# Autodesk Inventor assembly: Power Entry Module - Soanar PP4003
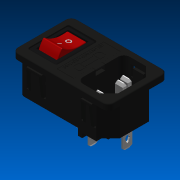
[picture p0: Inventor's stored thumbnail of the model, 180x180]
Saved by Autodesk Inventor 2016 (Build 200138000, 138)
## iProperties
Created: 2013-08-06
Document SubType Name: Assembly
Designer: sdarley
Project: Power Entry Module - Soanar PP4003
Catalog Web Link: https://www.soanarplus.com/getProductWebDetails.do?prodId=PP4003
Description: POWER ENTRY MODULE - SOANAR PP4003
Vendor: Soanar
Stock Number: PP4003
Author: sdarley
Title: Power Entry Module - Soanar PP4003
Revision Number: 1
## Documents named in this file (10)
- C:\Users\PowerStation9000\AppData\Local\Autodesk\Autodesk Sync\Cloud\mathiaslk\UltiBot mk2 rev2\Importerede komponenter\Power connector\Power Entry Module - Soanar PP4003.iam
- C:\Users\PowerStation9000\AppData\Local\Autodesk\Autodesk Sync\Cloud\mathiaslk\UltiBot mk2 rev2\Importerede komponenter\Power connector\Components\Rocker Switch - Arcolectric H8550VB\Rocker Switch - Arcolectric H8550VB.iam
- C:\Users\PowerStation9000\AppData\Local\Autodesk\Autodesk Sync\Cloud\mathiaslk\UltiBot mk2 rev2\Importerede komponenter\Power connector\Components\Soanar Power Module Fuse Cover.ipt
- C:\Users\PowerStation9000\AppData\Local\Autodesk\Autodesk Sync\Cloud\mathiaslk\UltiBot mk2 rev2\Importerede komponenter\Power connector\Components\Soanar Power Module Housing.ipt
- C:\Users\PowerStation9000\AppData\Local\Autodesk\Autodesk Sync\Cloud\mathiaslk\UltiBot mk2 rev2\Importerede komponenter\Power connector\Components\Soanar Power Module Pin A.ipt
- C:\Users\PowerStation9000\AppData\Local\Autodesk\Autodesk Sync\Cloud\mathiaslk\UltiBot mk2 rev2\Importerede komponenter\Power connector\Components\Soanar Power Module Pin B.ipt
- C:\Users\PowerStation9000\AppData\Local\Autodesk\Autodesk Sync\Cloud\mathiaslk\UltiBot mk2 rev2\Importerede komponenter\Power connector\Components\Soanar Power Module Pin C.ipt
- C:\Users\PowerStation9000\AppData\Local\Autodesk\Autodesk Sync\Cloud\mathiaslk\UltiBot mk2 rev2\Importerede komponenter\Power connector\Components\Soanar Power Module Pin D.ipt
- C:\Users\PowerStation9000\AppData\Local\Autodesk\Autodesk Sync\Cloud\mathiaslk\UltiBot mk2 rev2\Importerede komponenter\Power connector\Components\Soanar Power Module Pin E.ipt
- C:\Users\PowerStation9000\AppData\Local\Autodesk\Autodesk Sync\Cloud\mathiaslk\UltiBot mk2 rev2\Importerede komponenter\Power connector\Components\Soanar Power Module Fuse Holder.ipt
## Components (12 placed, 9 different names)
1. Soanar Power Module Housing:1 — Mate:1, Flush:1, Flush:2, Mate:4, Flush:4, Flush:5, Mate:2, Mate:5, Flush:6, Flush:7, Mate:6, Mate:7, Mate:8, Flush:8, Mate:12, Flush:14, Mate:14, Mate:16, Flush:15, Flush:16, Mate:20, Mate:22, Mate:23
2. Soanar Power Module Fuse Cover:1 — Flush:4, Flush:5, Mate:2, Mate:24, Mate:25, Mate:26
3. Soanar Power Module Pin A:1 — Flush:6, Flush:7, Mate:6, Mate:11
4. Soanar Power Module Pin B:1 — Mate:8, Mate:9, Mate:10, Mate:11, Flush:8
5. Soanar Power Module Pin B:2 — Mate:7, Mate:9, Mate:10
6. Soanar Power Module Pin C:1 — Mate:15, Mate:16, Mate:17, Mate:18, Mate:19
7. Soanar Power Module Pin C:2 — Mate:12, Flush:14, Mate:14, Mate:15, Mate:17, Flush:17, Mate:21
8. Soanar Power Module Pin D:1 — Flush:15, Mate:18, Mate:19
9. Soanar Power Module Pin E:1 — Flush:16, Mate:20, Flush:17
10. Soanar Power Module Fuse Holder:1 — Mate:23, Mate:24, Flush:18, Mate:26
11. Soanar Power Module Fuse Holder:2 — Mate:22, Mate:25, Flush:18
12. Rocker Switch - Arcolectric H8550VB:1 [sub-assembly] — Mate:1, Mate:4, Mate:5
## Relationships (36: Mate 24, Flush 12)
- Mate:1: Soanar Power Module Housing:1 ↔ Rocker Switch - Arcolectric H8550VB:1
- Flush:1: Soanar Power Module Housing:1
- Flush:2: Soanar Power Module Housing:1
- Mate:4: Soanar Power Module Housing:1 ↔ Rocker Switch - Arcolectric H8550VB:1
- Flush:4: Soanar Power Module Housing:1 ↔ Soanar Power Module Fuse Cover:1
- Flush:5: Soanar Power Module Housing:1 ↔ Soanar Power Module Fuse Cover:1
- Mate:2: Soanar Power Module Housing:1 ↔ Soanar Power Module Fuse Cover:1
- Mate:5 (0.025 mm): Soanar Power Module Housing:1 ↔ Rocker Switch - Arcolectric H8550VB:1
- Flush:6: Soanar Power Module Housing:1 ↔ Soanar Power Module Pin A:1
- Flush:7: Soanar Power Module Housing:1 ↔ Soanar Power Module Pin A:1
- Mate:6 (3.85 mm): Soanar Power Module Housing:1 ↔ Soanar Power Module Pin A:1
- Mate:7: Soanar Power Module Housing:1 ↔ Soanar Power Module Pin B:2
- Mate:8: Soanar Power Module Housing:1 ↔ Soanar Power Module Pin B:1
- Mate:9: Soanar Power Module Pin B:1 ↔ Soanar Power Module Pin B:2
- Mate:10 (13.15 mm): Soanar Power Module Pin B:1 ↔ Soanar Power Module Pin B:2
- Mate:11: Soanar Power Module Pin A:1 ↔ Soanar Power Module Pin B:1
- Flush:8 (-6.575 mm): Soanar Power Module Housing:1 ↔ Soanar Power Module Pin B:1
- Mate:12: Soanar Power Module Housing:1 ↔ Soanar Power Module Pin C:2
- Flush:14 (3.45 mm): Soanar Power Module Housing:1 ↔ Soanar Power Module Pin C:2
- Mate:14: Soanar Power Module Housing:1 ↔ Soanar Power Module Pin C:2
- Mate:15 (-11.2 mm): Soanar Power Module Pin C:1 ↔ Soanar Power Module Pin C:2
- Mate:16: Soanar Power Module Housing:1 ↔ Soanar Power Module Pin C:1
- Mate:17 (-11.9 mm): Soanar Power Module Pin C:1 ↔ Soanar Power Module Pin C:2
- Flush:15: Soanar Power Module Housing:1 ↔ Soanar Power Module Pin D:1
- Mate:18 (-11.6 mm): Soanar Power Module Pin C:1 ↔ Soanar Power Module Pin D:1
- Mate:19 (-4.6 mm): Soanar Power Module Pin C:1 ↔ Soanar Power Module Pin D:1
- Flush:16: Soanar Power Module Housing:1 ↔ Soanar Power Module Pin E:1
- Mate:20 (-9.75 mm): Soanar Power Module Housing:1 ↔ Soanar Power Module Pin E:1
- Flush:17 (-23.95 mm): Soanar Power Module Pin C:2 ↔ Soanar Power Module Pin E:1
- Mate:21: Soanar Power Module Pin C:2
- Mate:22: Soanar Power Module Housing:1 ↔ Soanar Power Module Fuse Holder:2
- Mate:23: Soanar Power Module Housing:1 ↔ Soanar Power Module Fuse Holder:1
- Mate:24: Soanar Power Module Fuse Cover:1 ↔ Soanar Power Module Fuse Holder:1
- Mate:25: Soanar Power Module Fuse Cover:1 ↔ Soanar Power Module Fuse Holder:2
- Flush:18 (16.5 mm): Soanar Power Module Fuse Holder:1 ↔ Soanar Power Module Fuse Holder:2
- Mate:26 (8.25 mm): Soanar Power Module Fuse Cover:1 ↔ Soanar Power Module Fuse Holder:1
